# Autodesk Inventor assembly: FullAssembly
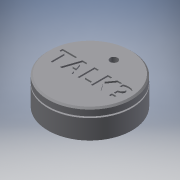
[picture p0: Inventor's stored thumbnail of the model, 180x180]
Saved by Autodesk Inventor 2019 (Build 230136000, 136)
## iProperties
Created: 2019-10-05
Part Number: FullAssembly
Document SubType Name: Assembly
Designer: Josiah
Author: Josiah
## iProperties of the stored document M2 Nut.ipt
Created: 2019-05-01
Part Number: M2 Nut
Material: Generic
Description: STEP AP214
Document SubType Name: Modeling
Designer: Josiah
Density: 1 g/cm^3
Appearance: Default
Sending System: SolidWorks 2018
Preprocessor: SwSTEP 2.0
Title: M2 Nut.STEP
Revision Number: HERHANGÝ
## Documents named in this file (9)
- **C:\Users\josia\OneDrive\Apps\MarksButtonC#\CAD\FullAssembly.iam*LocalDocs*xWzual1leQwoduicaZf43lp3x3a*M2 Nut.ipt
- C:\Users\josia\OneDrive\Apps\MarksButtonC#\CAD\FullAssembly.iam
- C:\Users\josia\OneDrive\Apps\MarksButtonC#\CAD\Base.ipt
- C:\Users\josia\OneDrive\Apps\MarksButtonC#\CAD\Imported Models\ArduinoNano\arduino nano.iam
- C:\Users\josia\OneDrive\Apps\MarksButtonC#\CAD\InternalSupportBracket.ipt
- C:\Users\josia\OneDrive\Apps\MarksButtonC#\CAD\Button.ipt
- C:\Users\josia\OneDrive\Apps\MarksButtonC#\CAD\ButtonCap.ipt
- C:\Users\josia\OneDrive\Apps\MarksButtonC#\CAD\Imported Models\M# Bolts\M2 x 0.4mm Thread 10mm LONG SOCKET HEAD CAP SCREW.ipt
- C:\Users\josia\OneDrive\Apps\MarksButtonC#\CAD\Imported Models\M# Nuts\M2 Nut.STEP
## Components (7 placed, 7 different names)
1. Base:1 — Mate:3, Mate:4, Mate:5, Mate:6, Mate:7, Mate:12, Mate:13, Mate:14, Mate:15, Mate:17, Mate:18, Mate:19
2. arduino nano:1 [sub-assembly] — Mate:3, Mate:4, Mate:17
3. InternalSupportBracket:1 — Mate:5, Mate:6, Mate:7, Mate:8, Flush:1, Flush:2
4. Button:1 — Mate:8, Flush:1, Flush:2, Mate:16
5. M2 Nut:1 — Mate:14, Mate:15
6. ButtonCap:1 — Mate:16, Mate:18, Mate:19
7. M2 x 0.4mm Thread 10mm LONG SOCKET HEAD CAP SCREW:1 — Mate:12, Mate:13
## Relationships (16: Mate 14, Flush 2)
- Mate:3: Base:1 ↔ arduino nano:1
- Mate:4: Base:1 ↔ arduino nano:1
- Mate:5: Base:1 ↔ InternalSupportBracket:1
- Mate:6: Base:1 ↔ InternalSupportBracket:1
- Mate:7: Base:1 ↔ InternalSupportBracket:1
- Mate:8: InternalSupportBracket:1 ↔ Button:1
- Flush:1 (12 mm): InternalSupportBracket:1 ↔ Button:1
- Flush:2 (-1.25 mm): InternalSupportBracket:1 ↔ Button:1
- Mate:12: Base:1 ↔ M2 x 0.4mm Thread 10mm LONG SOCKET HEAD CAP SCREW:1
- Mate:13: Base:1 ↔ M2 x 0.4mm Thread 10mm LONG SOCKET HEAD CAP SCREW:1
- Mate:14: Base:1 ↔ M2 Nut:1
- Mate:15 (0.1 mm): Base:1 ↔ M2 Nut:1
- Mate:16: Button:1 ↔ ButtonCap:1
- Mate:17: Base:1 ↔ arduino nano:1
- Mate:18: Base:1 ↔ ButtonCap:1
- Mate:19: Base:1 ↔ ButtonCap:1
